# Autodesk Inventor assembly: Fath 093P45LN Panel Holder
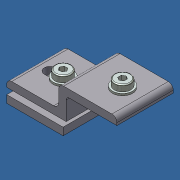
[picture p0: Inventor's stored thumbnail of the model, 180x180]
Saved by Autodesk Inventor 2012 (Build 160160000, 160)
## iProperties
Created: 2014-06-11
Part Number: Fath 093P45LN Panel Holder
Document SubType Name: Assembly
Designer: Mike Taylor
Mass: 136.969 g
Surface Area: 199.627 cm^2
Volume: 42.6979 cm^3
Density: 3.20786 g/cm^3
Author: Mike Taylor
## Documents named in this file (6)
- C:\Andys Backup Data\ANDY'S INVENTOR\INVENTOR LIBRARIES\PARTS LIBRARY\FITTING OF PANEL ELEMENTS ASSEMBLY POSSIBILITIES\21.9580 MESH FASTENER 45.iam
- C:\Andys Backup Data\ANDY'S INVENTOR\INVENTOR LIBRARIES\PARTS LIBRARY\FITTING OF PANEL ELEMENTS ASSEMBLY POSSIBILITIES\SUBCOMPONENTS\21.9580 MESH FASTENER 45 BRACKET.ipt
- C:\Andys Backup Data\ANDY'S INVENTOR\INVENTOR LIBRARIES\PARTS LIBRARY\FITTING OF PANEL ELEMENTS ASSEMBLY POSSIBILITIES\SUBCOMPONENTS\21.9580 MESH FASTENER 45 BACK PLATE.ipt
- C:\Andys Backup Data\ANDY'S INVENTOR\INVENTOR LIBRARIES\PARTS LIBRARY\FASTENING ELEMENTS\WASHERS\21.1127 M8 ROUND WASHER.ipt
- C:\Andys Backup Data\ANDY'S INVENTOR\INVENTOR LIBRARIES\PARTS LIBRARY\FASTENING ELEMENTS\SCREWS CAP\21.1202 M8X20.ipt
- C:\Andys Backup Data\ANDY'S INVENTOR\INVENTOR LIBRARIES\PARTS LIBRARY\FASTENING ELEMENTS\NUTS\21.1351_2 M8 SQUARE NUT POS FXG.ipt
## Components (7 placed, 5 different names)
1. 21.9580 MESH FASTENER 45 BRACKET:1 — Mate:1, Flush:1, Flush:2, Insert:1, Insert:5, Angle:1
2. 21.9580 MESH FASTENER 45 BACK PLATE:1 — Mate:1, Flush:1, Flush:2, Insert:2
3. 21.1127 WASHER M8:1 — Insert:1, Insert:3
4. 21.1127 WASHER M8:2 — Insert:2, Insert:4
5. 21.1202  M8 x 20:1 — Insert:3
6. 21.1202  M8 x 20:2 — Insert:4
7. 21.1351_2 M8 SQUARE NUT POS FXG:1 — Insert:5, Angle:1
## Relationships (9: Insert 5, Flush 2, Mate 1, Angle 1)
- Mate:1 (5.08 mm): 21.9580 MESH FASTENER 45 BRACKET:1 ↔ 21.9580 MESH FASTENER 45 BACK PLATE:1
- Flush:1: 21.9580 MESH FASTENER 45 BRACKET:1 ↔ 21.9580 MESH FASTENER 45 BACK PLATE:1
- Flush:2: 21.9580 MESH FASTENER 45 BRACKET:1 ↔ 21.9580 MESH FASTENER 45 BACK PLATE:1
- Insert:1: 21.9580 MESH FASTENER 45 BRACKET:1 ↔ 21.1127 WASHER M8:1
- Insert:2 (11.096 mm): 21.9580 MESH FASTENER 45 BACK PLATE:1 ↔ 21.1127 WASHER M8:2
- Insert:3: 21.1127 WASHER M8:1 ↔ 21.1202  M8 x 20:1
- Insert:4: 21.1127 WASHER M8:2 ↔ 21.1202  M8 x 20:2
- Insert:5 (4.5 mm): 21.9580 MESH FASTENER 45 BRACKET:1 ↔ 21.1351_2 M8 SQUARE NUT POS FXG:1
- Angle:1 (0 deg): 21.9580 MESH FASTENER 45 BRACKET:1 ↔ 21.1351_2 M8 SQUARE NUT POS FXG:1
